# Autodesk Inventor assembly: Hydraulikzylinder_Presse
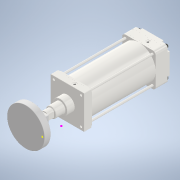
[picture p0: Inventor's stored thumbnail of the model, 180x180]
Saved by Autodesk Inventor 2020.3 (Build 243373000, 373)
## iProperties
Created: 2021-05-29
Part Number: Hydraulikzylinder_Presse
Document SubType Name: Assembly
Designer: Preuß P. Ch.
Author: Preuß P. Ch.
## Documents named in this file (10)
- D:\Studium\Praegemaschine\3D-Modelle\Hydraulikzylinder_Presse.iam
- C:\Users\user\Documents\Inventor\Hydraulikzylinder\Gehäuse.ipt
- C:\Users\user\Documents\Inventor\Hydraulikzylinder\Deckel_hinten.ipt
- C:\Users\user\Documents\Inventor\Hydraulikzylinder\Kolben.ipt
- C:\Users\user\Documents\Inventor\Hydraulikzylinder\Kolbenstange.ipt
- C:\Users\user\Documents\Inventor\Hydraulikzylinder\Deckel_vorne.ipt
- C:\Users\user\Documents\Inventor\Hydraulikzylinder\Gewindestange.ipt
- C:\Users\user\Documents\Inventor\Content Center Files\R2020\de-DE\ISO 4033(1)\ISO 4033 - M10DIN EN.ipt
- C:\Users\user\Documents\Inventor\Hydraulikzylinder\Gelenkflansch_Hinten_ohne_halterung.ipt
- C:\Users\user\Documents\Inventor\Hydraulikzylinder\Press_Stempel.ipt
## Components (19 placed, 9 different names)
1. Gehäuse:1 — Einfügen:1, Passend:1, Passend:5, Passend:8, Passend:9, Einfügen:9
2. Deckel_hinten:1 — Einfügen:1, Passend:1, Winkel:1, Verfahrweg, Winkel:2, Passend:12
3. Kolben:1 — Passend:5, Passend:6, Passend:7, Verfahrweg, Winkel:2, Unterdrücken_bei_Verfahrweg
4. Kolbenstange:1 — Passend:6, Passend:7, Winkel:1, Passend:14, Einfügen:10, Passend:15
5. Deckel_vorne:1 — Passend:8, Passend:9, Einfügen:6, Einfügen:7, Einfügen:8, Unterdrücken_bei_Verfahrweg
6. Gewindestange:1
7. Gewindestange:2 — Passend:13
8. Gewindestange:3
9. Gewindestange:4
10. Gelenkflansch_Hinten_ohne_halterung:1 — Passend:12, Passend:13
11. Press_Stempel:1 — Passend:14, Einfügen:10, Passend:15
12. DIN EN 24033 M10:1 — Einfügen:6
13. DIN EN 24033 M10:2 — Einfügen:7
14. DIN EN 24033 M10:3 — Einfügen:9
15. DIN EN 24033 M10:4 — Einfügen:8
16. DIN EN 24033 M10:5
17. DIN EN 24033 M10:6
18. DIN EN 24033 M10:7
19. DIN EN 24033 M10:8
## Relationships (20: Mate 12, Insert 6, Angle 2)
- Einfügen:1 [Insert]: Gehäuse:1 ↔ Deckel_hinten:1
- Passend:1 [Mate]: Gehäuse:1 ↔ Deckel_hinten:1
- Passend:5 [Mate]: Gehäuse:1 ↔ Kolben:1
- Passend:6 [Mate]: Kolben:1 ↔ Kolbenstange:1
- Passend:7 [Mate]: Kolben:1 ↔ Kolbenstange:1
- Winkel:1 [Angle] (0 deg): Deckel_hinten:1 ↔ Kolbenstange:1
- Passend:8 [Mate]: Gehäuse:1 ↔ Deckel_vorne:1
- Passend:9 [Mate]: Gehäuse:1 ↔ Deckel_vorne:1
- Verfahrweg [Mate]: Deckel_hinten:1 ↔ Kolben:1
- Winkel:2 [Angle] (0 deg): Deckel_hinten:1 ↔ Kolben:1
- Einfügen:6 [Insert]: Deckel_vorne:1 ↔ DIN EN 24033 M10:1
- Einfügen:7 [Insert]: Deckel_vorne:1 ↔ DIN EN 24033 M10:2
- Einfügen:8 [Insert]: Deckel_vorne:1 ↔ DIN EN 24033 M10:4
- Einfügen:9 [Insert]: Gehäuse:1 ↔ DIN EN 24033 M10:3
- Unterdrücken_bei_Verfahrweg [Mate] (228 mm): Kolben:1 ↔ Deckel_vorne:1
- Passend:12 [Mate]: Deckel_hinten:1 ↔ Gelenkflansch_Hinten_ohne_halterung:1
- Passend:13 [Mate]: Gewindestange:2 ↔ Gelenkflansch_Hinten_ohne_halterung:1
- Passend:14 [Mate]: Kolbenstange:1 ↔ Press_Stempel:1
- Einfügen:10 [Insert]: Kolbenstange:1 ↔ Press_Stempel:1
- Passend:15 [Mate] (30 mm): Kolbenstange:1 ↔ Press_Stempel:1
